# Autodesk Inventor assembly: Actuator 1.5
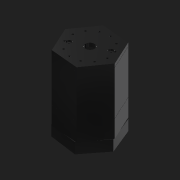
[picture p0: Inventor's stored thumbnail of the model, 180x180]
Saved by Autodesk Inventor 2017 (Build 210142000, 142)
## iProperties
Created: 2019-08-28
Part Number: Actuator 1.5
Document SubType Name: Assembly
Designer: Dell
Author: Dell
## Documents named in this file (13)
- C:\Users\Dell\Documents\GitHub\tr2\Actuator 1.5\Actuator 1.5.iam
- C:\Users\Dell\Documents\GitHub\tr2\Actuator 1.5\Slewing.iam
- C:\Users\Dell\Documents\GitHub\tr2\Actuator 1.5\AC01.ipt
- C:\Users\Dell\Documents\GitHub\tr2\Actuator 1.5\AC02.ipt
- C:\Users\Dell\Documents\GitHub\tr2\Actuator 1.5\12RPM Gear Motor.ipt
- C:\Users\Dell\Documents\GitHub\tr2\Actuator 1.5\AC03.ipt
- C:\Users\Dell\Documents\GitHub\tr2\Actuator 1.5\Actuator 1.5\Design Accelerator\Spur Gears1.iam
- C:\Users\Dell\Documents\GitHub\tr2\Actuator 1.5\6mm Mounting Hub, thick.ipt
- C:\Users\Dell\Documents\GitHub\tr2\Actuator 1.5\AEAT-6012.ipt
- C:\Users\Dell\Documents\GitHub\tr2\Actuator 1.5\AC04.ipt
- C:\Users\Dell\Documents\GitHub\tr2\Actuator 1.5\SEA Gearbox.iam
- C:\Users\Dell\Documents\GitHub\tr2\Actuator 1.5\Actuator 1.5\Design Accelerator\Spur Gears3.iam
- C:\Users\Dell\Documents\GitHub\tr2\Actuator 1.5\AC05.ipt
## Components (13 placed, 11 different names)
1. Slewing:1 [sub-assembly] — Mate:3, Mate:4, Mate:56, Mate:57, Mate:58, Mate:59
2. AC01:1 — Mate:3, Mate:4, Mate:23, Mate:35, Mate:50, Mate:59
3. AC02:1 — Mate:13, Mate:14, Mate:23, Mate:25, Mate:34, Mate:35, Mate:36, Mate:38, Mate:39, Mate:42, Mate:45, Mate:46, Mate:55, Mate:60
4. AC03:1
5. AC04:1 — Mate:42, Mate:45, Mate:46
6. AC05:1 — Mate:56, Mate:57
7. Spur Gears:4 [sub-assembly] — Mate:30, Mate:31, Mate:40
8. 12RPM Gear Motor:1 — Mate:13, Mate:14, Mate:24, Mate:34
9. 6mm Mounting Hub, thick:1 — Mate:24, Mate:25, Flush:1, Mate:30, Mate:31, Mate:40
10. 6mm Mounting Hub, thick:2 — Flush:1, Mate:36, Mate:54
11. AEAT-6012:1 — Mate:38, Mate:39, Mate:53, Mate:60
12. SEA Gearbox:1 [sub-assembly] — Mate:50, Mate:55, Mate:58
13. Spur Gears:5 [sub-assembly] — Mate:53, Mate:54
## Relationships (28: Mate 27, Flush 1)
- Mate:3: Slewing:1 ↔ AC01:1
- Mate:4: Slewing:1 ↔ AC01:1
- Mate:13: AC02:1 ↔ 12RPM Gear Motor:1
- Mate:14: AC02:1 ↔ 12RPM Gear Motor:1
- Mate:23: AC01:1 ↔ AC02:1
- Mate:24: 12RPM Gear Motor:1 ↔ 6mm Mounting Hub, thick:1
- Mate:25 (1 mm): AC02:1 ↔ 6mm Mounting Hub, thick:1
- Flush:1: 6mm Mounting Hub, thick:1 ↔ 6mm Mounting Hub, thick:2
- Mate:30: Spur Gears:4 ↔ 6mm Mounting Hub, thick:1
- Mate:31: Spur Gears:4 ↔ 6mm Mounting Hub, thick:1
- Mate:34: AC02:1 ↔ 12RPM Gear Motor:1
- Mate:35: AC01:1 ↔ AC02:1
- Mate:36: AC02:1 ↔ 6mm Mounting Hub, thick:2
- Mate:38: AC02:1 ↔ AEAT-6012:1
- Mate:39: AC02:1 ↔ AEAT-6012:1
- Mate:40: Spur Gears:4 ↔ 6mm Mounting Hub, thick:1
- Mate:42: AC02:1 ↔ AC04:1
- Mate:45: AC02:1 ↔ AC04:1
- Mate:46: AC02:1 ↔ AC04:1
- Mate:50: AC01:1 ↔ SEA Gearbox:1
- Mate:53: AEAT-6012:1 ↔ Spur Gears:5
- Mate:54: 6mm Mounting Hub, thick:2 ↔ Spur Gears:5
- Mate:55: AC02:1 ↔ SEA Gearbox:1
- Mate:56: Slewing:1 ↔ AC05:1
- Mate:57: Slewing:1 ↔ AC05:1
- Mate:58: Slewing:1 ↔ SEA Gearbox:1
- Mate:59: Slewing:1 ↔ AC01:1
- Mate:60: AC02:1 ↔ AEAT-6012:1
